# Autodesk Inventor assembly: perception module-01
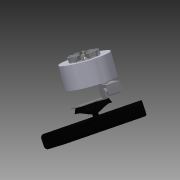
[picture p0: Inventor's stored thumbnail of the model, 180x180]
Saved by Autodesk Inventor 2015 (Build 190159000, 159)
## iProperties
Created: 2014-10-20
Part Number: perception module-01
Document SubType Name: Assembly
Designer: ericd_000
Author: ericd_000
## Documents named in this file (8)
- C:\Users\ericd_000\Dropbox\GitHub\initial_cad\eric_cad\perception module.iam
- C:\Users\ericd_000\Dropbox\GitHub\initial_cad\eric_cad\herkulex assembled.iam
- C:\Users\ericd_000\Dropbox\GitHub\initial_cad\eric_cad\per_base.ipt
- C:\Users\ericd_000\Dropbox\GitHub\initial_cad\eric_cad\first_perc_link.ipt
- C:\Users\ericd_000\Dropbox\GitHub\initial_cad\eric_cad\second_perc_link.ipt
- C:\Users\ericd_000\Dropbox\GitHub\initial_cad\eric_cad\male bayonet connector 12.ipt
- C:\Users\ericd_000\Dropbox\GitHub\initial_cad\eric_cad\Imported Components\kinect assembly\kinect assembly.iam
- perception module-01.iam
## Components (7 placed, 6 different names)
1. herkulex assembled:1 [sub-assembly] — Mate:2, Mate:3, Mate:4, Mate:10, Cylindrical:1
2. herkulex assembled:2 [sub-assembly] — Mate:7, Mate:8, Rotational:1, Flush:1
3. per_base:1 — Mate:5, Mate:6, Mate:7, Mate:8, Flush:1
4. first_perc_link:1 — Mate:2, Mate:10, Rotational:1, Cylindrical:1
5. second_perc_link:1 — Mate:3, Mate:4, Mate:11, Mate:12
6. male bayonet connector 12:1 — Mate:5, Mate:6
7. kinect assembly:1 [sub-assembly] — Mate:11, Mate:12
## Relationships (13: Mate 10, RevoluteJoint 1, Flush 1, CylindricalJoint 1)
- Mate:2: herkulex assembled:1 ↔ first_perc_link:1
- Mate:3: herkulex assembled:1 ↔ second_perc_link:1
- Mate:4: herkulex assembled:1 ↔ second_perc_link:1
- Mate:5: per_base:1 ↔ male bayonet connector 12:1
- Mate:6: per_base:1 ↔ male bayonet connector 12:1
- Mate:7 (5 mm): herkulex assembled:2 ↔ per_base:1
- Mate:8 (1 mm): herkulex assembled:2 ↔ per_base:1
- Mate:10: herkulex assembled:1 ↔ first_perc_link:1
- Rotational:1 [RevoluteJoint]: herkulex assembled:2 ↔ first_perc_link:1
- Flush:1 (-1 mm): herkulex assembled:2 ↔ per_base:1
- Cylindrical:1: herkulex assembled:1 ↔ first_perc_link:1
- Mate:11: second_perc_link:1 ↔ kinect assembly:1
- Mate:12 (0.2 mm): second_perc_link:1 ↔ kinect assembly:1
